# Autodesk Inventor assembly: Prototipo A
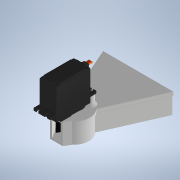
[picture p0: Inventor's stored thumbnail of the model, 180x180]
Saved by Autodesk Inventor 2020.3 (Build 243373000, 373)
## iProperties
Created: 2021-02-17
Part Number: Prototipo A
Document SubType Name: Assembly
Designer: juanp
Author: juanp
## Documents named in this file (5)
- C:\Users\juanp\Desktop\Robocol\Nuevo EVA\Prototipo 1\Prototipo 1.iam
- C:\Users\juanp\Desktop\Robocol\Nuevo EVA\Recursos\Servo MG996R\Servo Motor MG996R.iam
- C:\Users\juanp\Desktop\Robocol\Nuevo EVA\Prototipo 1\attachmentcustom.ipt
- C:\Users\juanp\Desktop\Robocol\Nuevo EVA\Prototipo 1\Valvula.ipt
- C:\Users\juanp\Desktop\Robocol\Nuevo EVA\Prototipo 1\embudo.ipt
## Components (4 placed, 4 different names)
1. Servo Motor MG996R:1 [sub-assembly] — Flush:2, Mate:2, Flush:4, Mate:4, Mate:5, Mate:8
2. attachmentcustom:1 — Mate:4, Mate:5, Mate:6, Flush:5, Mate:7, Flush:6
3. Valvula:1 — Mate:6, Flush:5
4. embudo:1 — Mate:7, Flush:6, Mate:8
## Relationships (10: Mate 6, Flush 4)
- Flush:2: Servo Motor MG996R:1
- Mate:2: Servo Motor MG996R:1
- Flush:4: Servo Motor MG996R:1
- Mate:4: Servo Motor MG996R:1 ↔ attachmentcustom:1
- Mate:5: Servo Motor MG996R:1 ↔ attachmentcustom:1
- Mate:6: attachmentcustom:1 ↔ Valvula:1
- Flush:5 (3 mm): attachmentcustom:1 ↔ Valvula:1
- Mate:7: attachmentcustom:1 ↔ embudo:1
- Flush:6: attachmentcustom:1 ↔ embudo:1
- Mate:8: Servo Motor MG996R:1 ↔ embudo:1
